# Autodesk Inventor assembly: 長穴減速_ホーン
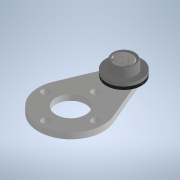
[picture p0: Inventor's stored thumbnail of the model, 180x180]
Saved by Autodesk Inventor 2020 (Build 240168000, 168)
## iProperties
Created: 2021-09-06
Part Number: 長穴減速_ホーン
Document SubType Name: Assembly
Designer: Masato
Author: Masato
## Documents named in this file (5)
- C:\Users\Masato\Documents\Inventor\CIT Brains_Inventor\OpenPlatform_ver3_0\下半身\長穴減速\長穴減速_ホーン.iam
- C:\Users\Masato\Documents\Inventor\CIT Brains_Inventor\OpenPlatform_ver3_0\下半身\長穴減速\長穴減速_ホーン_1.ipt
- C:\Users\Masato\Documents\Inventor\CIT Brains_Inventor\OpenPlatform_ver3_0\既製品\80F-0603.ipt
- C:\Users\Masato\Documents\Inventor\CIT Brains_Inventor\OpenPlatform_ver3_0\既製品\ARU-305S.ipt
- C:\Users\Masato\Documents\Inventor\CIT Brains_Inventor\OpenPlatform_ver3_0\既製品\CC-0612-10B.ipt
## Components (4 placed, 4 different names)
1. 長穴減速_ホーン_1:1 — 挿入:1
2. 80F-0603:1 — 挿入:3
3. ARU-305S:1 — 挿入:1, 挿入:2
4. CC-0612-10B:1 — 挿入:2, 挿入:3
## Relationships (3: Insert 3)
- 挿入:1 [Insert]: 長穴減速_ホーン_1:1 ↔ ARU-305S:1
- 挿入:2 [Insert]: ARU-305S:1 ↔ CC-0612-10B:1
- 挿入:3 [Insert]: 80F-0603:1 ↔ CC-0612-10B:1
